# Autodesk Inventor assembly: Ankle_front_frame
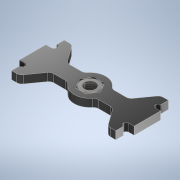
[picture p0: Inventor's stored thumbnail of the model, 180x180]
Saved by Autodesk Inventor 2022.3 (Build 263350000, 350)
## iProperties
Created: 2023-05-14
Part Number: Ankle_front_frame
Document SubType Name: Assembly
Designer: Masato Kubotera
Author: Masato Kubotera
## Documents named in this file (3)
- C:\Users\Masato\Documents\Inventor\Inventor for CIT Brains\SUSTAINA-OP - ankle\LowerBody\Ankle\Ankle_front_frame.iam
- C:\Users\Masato\Documents\Inventor\Inventor for CIT Brains\SUSTAINA-OP - ankle\LowerBody\Ankle\Ankle_front_frame.ipt
- C:\Users\Masato\Documents\Inventor\Inventor for CIT Brains\SUSTAINA-OP - ankle\ReadyMade\InsertNut\S4-05-3W.ipt
## Components (2 placed, 2 different names)
1. Ankle_front_frame:1 — フラッシュ:1, フラッシュ:2, フラッシュ:3, 挿入:1, 角度:1
2. S4-05-3W:1 — 挿入:1, 角度:1
## Relationships (5: Flush 3, Insert 1, Angle 1)
- フラッシュ:1 [Flush]: Ankle_front_frame:1
- フラッシュ:2 [Flush]: Ankle_front_frame:1
- フラッシュ:3 [Flush]: Ankle_front_frame:1
- 挿入:1 [Insert]: Ankle_front_frame:1 ↔ S4-05-3W:1
- 角度:1 [Angle] (0 deg): Ankle_front_frame:1 ↔ S4-05-3W:1
